# Autodesk Inventor assembly: Pi Case Assembly V 01
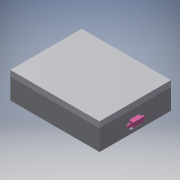
[picture p0: Inventor's stored thumbnail of the model, 180x180]
Saved by Autodesk Inventor 2016 (Build 200138000, 138)
## iProperties
Created: 2015-03-20
Part Number: Pi Case Assembly V 01
Document SubType Name: Assembly
Designer: steele
Author: steele
## Documents named in this file (7)
- C:\snobotics\CAD-Development\robSteele\RaspberryPi\Pi Case Assembly V 01.iam
- C:\snobotics\CAD-Development\robSteele\RaspberryPi\Pi Case Bottom V 01.ipt
- C:\snobotics\CAD-Development\robSteele\RaspberryPi\Vilros Pi Case.ipt
- C:\snobotics\CAD-Development\robSteele\RaspberryPi\RS 232 Board.ipt
- C:\snobotics\CAD-Development\robSteele\RaspberryPi\Pi Case Top V 01.ipt
- C:\snobotics\CAD-Development\robSteele\RaspberryPi\Pi Case Assembly V 01\Design Accelerator\Bolted Connection2.iam
- C:\snobotics\CAD-Development\robSteele\RaspberryPi\Pi Case Assembly V 01\Design Accelerator\Bolted Connection1.iam
## Components (7 placed, 5 different names)
1. Pi Case Bottom V 01:1 — Mate:1, Mate:2, Mate:3, Mate:4, Mate:5, Mate:6, Mate:7, Flush:1, Flush:2, Flush:3, Flush:4, Mate:12
2. Vilros Pi Case:1 — Mate:1, Mate:2, Mate:3
3. RS 232 Board:1 — Mate:4, Mate:5, Mate:6, Mate:8, Mate:9, Mate:10, Mate:11
4. Pi Case Top V 01:1 — Mate:7, Flush:1, Flush:2
5. Bolted Connection:1 [sub-assembly] — Mate:8, Mate:9
6. Bolted Connection:2 [sub-assembly] — Mate:10, Mate:11
7. Pi Case Top V 01:2 — Flush:3, Flush:4, Mate:12
## Relationships (16: Mate 12, Flush 4)
- Mate:1: Pi Case Bottom V 01:1 ↔ Vilros Pi Case:1
- Mate:2: Pi Case Bottom V 01:1 ↔ Vilros Pi Case:1
- Mate:3 (26.25 mm): Pi Case Bottom V 01:1 ↔ Vilros Pi Case:1
- Mate:4: Pi Case Bottom V 01:1 ↔ RS 232 Board:1
- Mate:5: Pi Case Bottom V 01:1 ↔ RS 232 Board:1
- Mate:6 (41.5 mm): Pi Case Bottom V 01:1 ↔ RS 232 Board:1
- Mate:7: Pi Case Bottom V 01:1 ↔ Pi Case Top V 01:1
- Flush:1: Pi Case Bottom V 01:1 ↔ Pi Case Top V 01:1
- Flush:2: Pi Case Bottom V 01:1 ↔ Pi Case Top V 01:1
- Mate:8: RS 232 Board:1 ↔ Bolted Connection:1
- Mate:9: RS 232 Board:1 ↔ Bolted Connection:1
- Mate:10: RS 232 Board:1 ↔ Bolted Connection:2
- Mate:11: RS 232 Board:1 ↔ Bolted Connection:2
- Flush:3: Pi Case Bottom V 01:1 ↔ Pi Case Top V 01:2
- Flush:4: Pi Case Bottom V 01:1 ↔ Pi Case Top V 01:2
- Mate:12: Pi Case Bottom V 01:1 ↔ Pi Case Top V 01:2
